# Autodesk Inventor assembly: strut_assem_LH
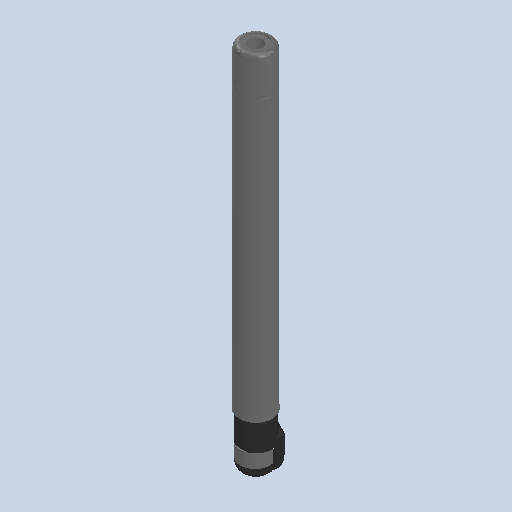
[picture p0: Inventor's stored thumbnail of the model, 512x512]
Saved by Autodesk Inventor 2024 (Build 280153000, 153)
## iProperties
Created: 2019-04-24
Part Number: strut_assem_LH
Document SubType Name: Assembly
Designer: Ishaan
Sending System: SolidWorks 2018
Last Author: Daniel Angeles
Last Saved: 2019-04-24
Author: Ishaan
## Documents named in this file (3)
- E:\Projects\Axiom--IDEX-3D-Printer\CAD\00 - COTS Components\Gas Strut Hardware\strut_assem\strut_assem_LH.iam
- E:\Projects\Axiom--IDEX-3D-Printer\CAD\00 - COTS Components\Gas Strut Hardware\strut_assem\base.ipt
- E:\Projects\Axiom--IDEX-3D-Printer\CAD\00 - COTS Components\Gas Strut Hardware\strut_assem\end_mounts.ipt
## Components (2 placed, 2 different names)
1. base:1 — Insert:2
2. end_mounts:1 — Insert:2
## Relationships (1: Insert 1)
- Insert:2: base:1 ↔ end_mounts:1
